# Autodesk Inventor assembly: 조립
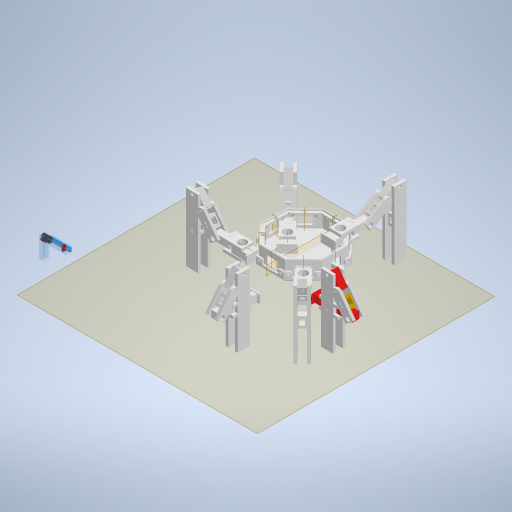
[picture p0: Inventor's stored thumbnail of the model, 512x512]
Saved by Autodesk Inventor 2024 (Build 280153000, 153)
## iProperties
Created: 2024-09-11
Part Number: 조립
Document SubType Name: Assembly
Designer: USER
Author: USER
## Documents named in this file (10)
- C:\Users\USER\Desktop\졸업작품\다리\조립.iam
- C:\Users\USER\Desktop\졸업작품\다리\다리 연결 부품-3.ipt
- C:\Users\USER\Desktop\졸업작품\다리\다리 프레임-0.ipt
- C:\Users\USER\Desktop\졸업작품\다리\다리 프레임-1.ipt
- C:\Users\USER\Desktop\졸업작품\다리\다리 프레임-2.ipt
- C:\Users\USER\Desktop\졸업작품\다리\다리 프레임-3.ipt
- C:\Users\USER\Desktop\졸업작품\다리\leg\LegTest.iam
- C:\Users\USER\Desktop\졸업작품\모터\모터.ipt
- C:\Users\USER\Desktop\졸업작품\다리\몸통.ipt
- C:\Users\USER\Desktop\졸업작품\다리\벽.ipt
## Components (76 placed, 9 different names)
1. 다리 연결 부품-3:1 — 메이트:12, 메이트:13, 메이트:14, 메이트:15, 메이트:25
2. 다리 프레임-0:1 — 메이트:3, 메이트:4, 메이트:11
3. 다리 프레임-1:1 — 메이트:3, 메이트:11, 메이트:16, 메이트:17, 메이트:39
4. 다리 프레임-2:1 — 메이트:12, 메이트:13, 메이트:22, 메이트:23, 메이트:25, 메이트:44, 메이트:46, 메이트:47
5. 다리 프레임-3:1 — 메이트:26, 메이트:27, 메이트:28, 메이트:48
6. 다리 프레임-1:2 — 메이트:4, 메이트:18, 메이트:19, 메이트:20
7. LegTest:1 [sub-assembly]
8. 모터:2 — 메이트:16, 메이트:17, 메이트:18, 메이트:19, 메이트:20, 메이트:21, 메이트:22, 메이트:23, 메이트:24, 메이트:39
9. 다리 프레임-2:2 — 메이트:14, 메이트:15, 메이트:21, 메이트:24
10. 다리 연결 부품-3:2 — 메이트:26, 메이트:27, 메이트:28, 메이트:29, 메이트:30, 메이트:31
11. 다리 프레임-3:2 — 메이트:29, 메이트:30, 메이트:31, 메이트:42, 메이트:45
12. 모터:3 — 메이트:42, 메이트:44, 메이트:45, 메이트:46, 메이트:47
13. 다리 연결 부품-3:3
14. 다리 프레임-0:2 — 메이트:208, 메이트:230, 메이트:231, 메이트:232
15. 다리 프레임-1:3 — 메이트:208
16. 다리 프레임-2:3
17. 다리 프레임-3:3 — 메이트:201
18. 다리 프레임-1:4
19. 모터:4
20. 다리 프레임-2:4
21. 다리 연결 부품-3:4
22. 다리 프레임-3:4
23. 모터:5
24. 다리 연결 부품-3:5
25. 다리 프레임-0:3
26. 다리 프레임-1:5
27. 다리 프레임-2:5
28. 다리 프레임-3:5 — 메이트:202, 메이트:206
29. 다리 프레임-1:6
30. 모터:6
31. 다리 프레임-2:6
32. 다리 연결 부품-3:6
33. 다리 프레임-3:6
34. 모터:7
35. 다리 연결 부품-3:7
36. 다리 프레임-0:4 — 메이트:211
37. 다리 프레임-1:7 — 메이트:211
38. 다리 프레임-2:7
39. 다리 프레임-3:7
40. 다리 프레임-1:8
41. 모터:8
42. 다리 프레임-2:8
43. 다리 연결 부품-3:8
44. 다리 프레임-3:8 — 메이트:204
45. 모터:9
46. 다리 연결 부품-3:9
47. 다리 프레임-0:5 — 메이트:212
48. 다리 프레임-1:9 — 메이트:212
49. 다리 프레임-2:9
50. 다리 프레임-3:9
51. 다리 프레임-1:10
52. 모터:10
53. 다리 프레임-2:10
54. 다리 연결 부품-3:10
55. 다리 프레임-3:10 — 메이트:203
56. 모터:11
57. 다리 연결 부품-3:11
58. 다리 프레임-0:6
59. 다리 프레임-1:11
60. 다리 프레임-2:11
61. 다리 프레임-3:11
62. 다리 프레임-1:12
63. 모터:12
64. 다리 프레임-2:12
65. 다리 연결 부품-3:12
66. 다리 프레임-3:12 — 메이트:205
67. 모터:13
68. 몸통:1 — 메이트:214, 메이트:215, 메이트:223, 메이트:224, 메이트:225, 메이트:226, 메이트:227, 메이트:228, 메이트:229, 플러쉬:8
69. 벽:1 — 메이트:214, 메이트:215, 메이트:216, 플러쉬:1
70. 벽:2 — 메이트:216, 플러쉬:1, 메이트:217, 플러쉬:2, 메이트:223
71. 벽:3 — 메이트:217, 플러쉬:2, 메이트:218, 플러쉬:3, 메이트:224
72. 벽:4 — 메이트:219, 플러쉬:4, 메이트:220, 플러쉬:5, 메이트:226
73. 벽:5 — 메이트:220, 플러쉬:5, 메이트:221, 플러쉬:6, 메이트:227, 플러쉬:8
74. 벽:6 — 메이트:218, 플러쉬:3, 메이트:219, 플러쉬:4, 메이트:225
75. 벽:7 — 메이트:221, 플러쉬:6, 메이트:222, 플러쉬:7, 메이트:228, 메이트:230, 메이트:231, 메이트:232
76. 벽:8 — 메이트:222, 플러쉬:7, 메이트:229
## Relationships (211: Mate 203, Flush 8)
- 메이트:3 [Mate]: 다리 프레임-0:1 ↔ 다리 프레임-1:1
- 메이트:4 [Mate]: 다리 프레임-0:1 ↔ 다리 프레임-1:2
- 메이트:11 [Mate]: 다리 프레임-0:1 ↔ 다리 프레임-1:1
- 메이트:12 [Mate]: 다리 연결 부품-3:1 ↔ 다리 프레임-2:1
- 메이트:13 [Mate]: 다리 연결 부품-3:1 ↔ 다리 프레임-2:1
- 메이트:14 [Mate]: 다리 연결 부품-3:1 ↔ 다리 프레임-2:2
- 메이트:15 [Mate]: 다리 연결 부품-3:1 ↔ 다리 프레임-2:2
- 메이트:16 [Mate]: 다리 프레임-1:1 ↔ 모터:2
- 메이트:17 [Mate]: 다리 프레임-1:1 ↔ 모터:2
- 메이트:18 [Mate]: 다리 프레임-1:2 ↔ 모터:2
- 메이트:19 [Mate]: 다리 프레임-1:2 ↔ 모터:2
- 메이트:20 [Mate]: 다리 프레임-1:2 ↔ 모터:2
- 메이트:21 [Mate]: 모터:2 ↔ 다리 프레임-2:2
- 메이트:22 [Mate]: 다리 프레임-2:1 ↔ 모터:2
- 메이트:23 [Mate]: 다리 프레임-2:1 ↔ 모터:2
- 메이트:24 [Mate]: 모터:2 ↔ 다리 프레임-2:2
- 메이트:25 [Mate]: 다리 연결 부품-3:1 ↔ 다리 프레임-2:1
- 메이트:26 [Mate]: 다리 프레임-3:1 ↔ 다리 연결 부품-3:2
- 메이트:27 [Mate]: 다리 프레임-3:1 ↔ 다리 연결 부품-3:2
- 메이트:28 [Mate]: 다리 프레임-3:1 ↔ 다리 연결 부품-3:2
- 메이트:29 [Mate]: 다리 연결 부품-3:2 ↔ 다리 프레임-3:2
- 메이트:30 [Mate]: 다리 연결 부품-3:2 ↔ 다리 프레임-3:2
- 메이트:31 [Mate]: 다리 연결 부품-3:2 ↔ 다리 프레임-3:2
- 메이트:39 [Mate]: 다리 프레임-1:1 ↔ 모터:2
- 메이트:42 [Mate]: 다리 프레임-3:2 ↔ 모터:3
- 메이트:44 [Mate]: 다리 프레임-2:1 ↔ 모터:3
- 메이트:45 [Mate]: 다리 프레임-3:2 ↔ 모터:3
- 메이트:46 [Mate]: 다리 프레임-2:1 ↔ 모터:3
- 메이트:47 [Mate]: 다리 프레임-2:1 ↔ 모터:3
- 메이트:48 [Mate]: 다리 프레임-3:1
- [Mate]: 다리 프레임-0:2 ↔ 다리 프레임-1:3
- [Mate]: 다리 프레임-0:2 ↔ 다리 프레임-1:4
- [Mate]: 다리 프레임-0:2 ↔ 다리 프레임-1:3
- [Mate]: 다리 연결 부품-3:3 ↔ 다리 프레임-2:3
- [Mate]: 다리 연결 부품-3:3 ↔ 다리 프레임-2:3
- [Mate]: 다리 연결 부품-3:3 ↔ 다리 프레임-2:4
- [Mate]: 다리 연결 부품-3:3 ↔ 다리 프레임-2:4
- [Mate]: 다리 프레임-1:3 ↔ 모터:4
- [Mate]: 다리 프레임-1:3 ↔ 모터:4
- [Mate]: 다리 프레임-1:4 ↔ 모터:4
- [Mate]: 다리 프레임-1:4 ↔ 모터:4
- [Mate]: 다리 프레임-1:4 ↔ 모터:4
- [Mate]: 모터:4 ↔ 다리 프레임-2:4
- [Mate]: 다리 프레임-2:3 ↔ 모터:4
- [Mate]: 다리 프레임-2:3 ↔ 모터:4
- [Mate]: 모터:4 ↔ 다리 프레임-2:4
- [Mate]: 다리 연결 부품-3:3 ↔ 다리 프레임-2:3
- [Mate]: 다리 프레임-3:3 ↔ 다리 연결 부품-3:4
- [Mate]: 다리 프레임-3:3 ↔ 다리 연결 부품-3:4
- [Mate]: 다리 프레임-3:3 ↔ 다리 연결 부품-3:4
- [Mate]: 다리 연결 부품-3:4 ↔ 다리 프레임-3:4
- [Mate]: 다리 연결 부품-3:4 ↔ 다리 프레임-3:4
- [Mate]: 다리 연결 부품-3:4 ↔ 다리 프레임-3:4
- [Mate]: 다리 프레임-1:3 ↔ 모터:4
- [Mate]: 다리 프레임-3:4 ↔ 모터:5
- [Mate]: 다리 프레임-2:3 ↔ 모터:5
- [Mate]: 다리 프레임-3:4 ↔ 모터:5
- [Mate]: 다리 프레임-2:3 ↔ 모터:5
- [Mate]: 다리 프레임-2:3 ↔ 모터:5
- [Mate]: 다리 프레임-0:3 ↔ 다리 프레임-1:5
- [Mate]: 다리 프레임-0:3 ↔ 다리 프레임-1:6
- [Mate]: 다리 프레임-0:3 ↔ 다리 프레임-1:5
- [Mate]: 다리 연결 부품-3:5 ↔ 다리 프레임-2:5
- [Mate]: 다리 연결 부품-3:5 ↔ 다리 프레임-2:5
- [Mate]: 다리 연결 부품-3:5 ↔ 다리 프레임-2:6
- [Mate]: 다리 연결 부품-3:5 ↔ 다리 프레임-2:6
- [Mate]: 다리 프레임-1:5 ↔ 모터:6
- [Mate]: 다리 프레임-1:5 ↔ 모터:6
- [Mate]: 다리 프레임-1:6 ↔ 모터:6
- [Mate]: 다리 프레임-1:6 ↔ 모터:6
- [Mate]: 다리 프레임-1:6 ↔ 모터:6
- [Mate]: 모터:6 ↔ 다리 프레임-2:6
- [Mate]: 다리 프레임-2:5 ↔ 모터:6
- [Mate]: 다리 프레임-2:5 ↔ 모터:6
- [Mate]: 모터:6 ↔ 다리 프레임-2:6
- [Mate]: 다리 연결 부품-3:5 ↔ 다리 프레임-2:5
- [Mate]: 다리 프레임-3:5 ↔ 다리 연결 부품-3:6
- [Mate]: 다리 프레임-3:5 ↔ 다리 연결 부품-3:6
- [Mate]: 다리 프레임-3:5 ↔ 다리 연결 부품-3:6
- [Mate]: 다리 연결 부품-3:6 ↔ 다리 프레임-3:6
- [Mate]: 다리 연결 부품-3:6 ↔ 다리 프레임-3:6
- [Mate]: 다리 연결 부품-3:6 ↔ 다리 프레임-3:6
- [Mate]: 다리 프레임-1:5 ↔ 모터:6
- [Mate]: 다리 프레임-3:6 ↔ 모터:7
- [Mate]: 다리 프레임-2:5 ↔ 모터:7
- [Mate]: 다리 프레임-3:6 ↔ 모터:7
- [Mate]: 다리 프레임-2:5 ↔ 모터:7
- [Mate]: 다리 프레임-2:5 ↔ 모터:7
- [Mate]: 다리 프레임-0:4 ↔ 다리 프레임-1:7
- [Mate]: 다리 프레임-0:4 ↔ 다리 프레임-1:8
- [Mate]: 다리 프레임-0:4 ↔ 다리 프레임-1:7
- [Mate]: 다리 연결 부품-3:7 ↔ 다리 프레임-2:7
- [Mate]: 다리 연결 부품-3:7 ↔ 다리 프레임-2:7
- [Mate]: 다리 연결 부품-3:7 ↔ 다리 프레임-2:8
- [Mate]: 다리 연결 부품-3:7 ↔ 다리 프레임-2:8
- [Mate]: 다리 프레임-1:7 ↔ 모터:8
- [Mate]: 다리 프레임-1:7 ↔ 모터:8
- [Mate]: 다리 프레임-1:8 ↔ 모터:8
- [Mate]: 다리 프레임-1:8 ↔ 모터:8
- [Mate]: 다리 프레임-1:8 ↔ 모터:8
- [Mate]: 모터:8 ↔ 다리 프레임-2:8
- [Mate]: 다리 프레임-2:7 ↔ 모터:8
- [Mate]: 다리 프레임-2:7 ↔ 모터:8
- [Mate]: 모터:8 ↔ 다리 프레임-2:8
- [Mate]: 다리 연결 부품-3:7 ↔ 다리 프레임-2:7
- [Mate]: 다리 프레임-3:7 ↔ 다리 연결 부품-3:8
- [Mate]: 다리 프레임-3:7 ↔ 다리 연결 부품-3:8
- [Mate]: 다리 프레임-3:7 ↔ 다리 연결 부품-3:8
- [Mate]: 다리 연결 부품-3:8 ↔ 다리 프레임-3:8
- [Mate]: 다리 연결 부품-3:8 ↔ 다리 프레임-3:8
- [Mate]: 다리 연결 부품-3:8 ↔ 다리 프레임-3:8
- [Mate]: 다리 프레임-1:7 ↔ 모터:8
- [Mate]: 다리 프레임-3:8 ↔ 모터:9
- [Mate]: 다리 프레임-2:7 ↔ 모터:9
- [Mate]: 다리 프레임-3:8 ↔ 모터:9
- [Mate]: 다리 프레임-2:7 ↔ 모터:9
- [Mate]: 다리 프레임-2:7 ↔ 모터:9
- [Mate]: 다리 프레임-0:5 ↔ 다리 프레임-1:9
- [Mate]: 다리 프레임-0:5 ↔ 다리 프레임-1:10
- [Mate]: 다리 프레임-0:5 ↔ 다리 프레임-1:9
- [Mate]: 다리 연결 부품-3:9 ↔ 다리 프레임-2:9
- [Mate]: 다리 연결 부품-3:9 ↔ 다리 프레임-2:9
- [Mate]: 다리 연결 부품-3:9 ↔ 다리 프레임-2:10
- [Mate]: 다리 연결 부품-3:9 ↔ 다리 프레임-2:10
- [Mate]: 다리 프레임-1:9 ↔ 모터:10
- [Mate]: 다리 프레임-1:9 ↔ 모터:10
- [Mate]: 다리 프레임-1:10 ↔ 모터:10
- [Mate]: 다리 프레임-1:10 ↔ 모터:10
- [Mate]: 다리 프레임-1:10 ↔ 모터:10
- [Mate]: 모터:10 ↔ 다리 프레임-2:10
- [Mate]: 다리 프레임-2:9 ↔ 모터:10
- [Mate]: 다리 프레임-2:9 ↔ 모터:10
- [Mate]: 모터:10 ↔ 다리 프레임-2:10
- [Mate]: 다리 연결 부품-3:9 ↔ 다리 프레임-2:9
- [Mate]: 다리 프레임-3:9 ↔ 다리 연결 부품-3:10
- [Mate]: 다리 프레임-3:9 ↔ 다리 연결 부품-3:10
- [Mate]: 다리 프레임-3:9 ↔ 다리 연결 부품-3:10
- [Mate]: 다리 연결 부품-3:10 ↔ 다리 프레임-3:10
- [Mate]: 다리 연결 부품-3:10 ↔ 다리 프레임-3:10
- [Mate]: 다리 연결 부품-3:10 ↔ 다리 프레임-3:10
- [Mate]: 다리 프레임-1:9 ↔ 모터:10
- [Mate]: 다리 프레임-3:10 ↔ 모터:11
- [Mate]: 다리 프레임-2:9 ↔ 모터:11
- [Mate]: 다리 프레임-3:10 ↔ 모터:11
- [Mate]: 다리 프레임-2:9 ↔ 모터:11
- [Mate]: 다리 프레임-2:9 ↔ 모터:11
- [Mate]: 다리 프레임-0:6 ↔ 다리 프레임-1:11
- [Mate]: 다리 프레임-0:6 ↔ 다리 프레임-1:12
- [Mate]: 다리 프레임-0:6 ↔ 다리 프레임-1:11
- [Mate]: 다리 연결 부품-3:11 ↔ 다리 프레임-2:11
- [Mate]: 다리 연결 부품-3:11 ↔ 다리 프레임-2:11
- [Mate]: 다리 연결 부품-3:11 ↔ 다리 프레임-2:12
- [Mate]: 다리 연결 부품-3:11 ↔ 다리 프레임-2:12
- [Mate]: 다리 프레임-1:11 ↔ 모터:12
- [Mate]: 다리 프레임-1:11 ↔ 모터:12
- [Mate]: 다리 프레임-1:12 ↔ 모터:12
- [Mate]: 다리 프레임-1:12 ↔ 모터:12
- [Mate]: 다리 프레임-1:12 ↔ 모터:12
- [Mate]: 모터:12 ↔ 다리 프레임-2:12
- [Mate]: 다리 프레임-2:11 ↔ 모터:12
- [Mate]: 다리 프레임-2:11 ↔ 모터:12
- [Mate]: 모터:12 ↔ 다리 프레임-2:12
- [Mate]: 다리 연결 부품-3:11 ↔ 다리 프레임-2:11
- [Mate]: 다리 프레임-3:11 ↔ 다리 연결 부품-3:12
- [Mate]: 다리 프레임-3:11 ↔ 다리 연결 부품-3:12
- [Mate]: 다리 프레임-3:11 ↔ 다리 연결 부품-3:12
- [Mate]: 다리 연결 부품-3:12 ↔ 다리 프레임-3:12
- [Mate]: 다리 연결 부품-3:12 ↔ 다리 프레임-3:12
- [Mate]: 다리 연결 부품-3:12 ↔ 다리 프레임-3:12
- [Mate]: 다리 프레임-1:11 ↔ 모터:12
- [Mate]: 다리 프레임-3:12 ↔ 모터:13
- [Mate]: 다리 프레임-2:11 ↔ 모터:13
- [Mate]: 다리 프레임-3:12 ↔ 모터:13
- [Mate]: 다리 프레임-2:11 ↔ 모터:13
- [Mate]: 다리 프레임-2:11 ↔ 모터:13
- 메이트:201 [Mate]: 다리 프레임-3:3
- 메이트:202 [Mate]: 다리 프레임-3:5
- 메이트:203 [Mate]: 다리 프레임-3:10
- 메이트:204 [Mate]: 다리 프레임-3:8
- 메이트:205 [Mate]: 다리 프레임-3:12
- 메이트:206 [Mate]: 다리 프레임-3:5
- 메이트:208 [Mate]: 다리 프레임-0:2 ↔ 다리 프레임-1:3
- 메이트:211 [Mate]: 다리 프레임-0:4 ↔ 다리 프레임-1:7
- 메이트:212 [Mate]: 다리 프레임-0:5 ↔ 다리 프레임-1:9
- 메이트:214 [Mate]: 몸통:1 ↔ 벽:1
- 메이트:215 [Mate]: 몸통:1 ↔ 벽:1
- 메이트:216 [Mate]: 벽:1 ↔ 벽:2
- 플러쉬:1 [Flush]: 벽:1 ↔ 벽:2
- 메이트:217 [Mate]: 벽:2 ↔ 벽:3
- 플러쉬:2 [Flush]: 벽:2 ↔ 벽:3
- 메이트:218 [Mate]: 벽:3 ↔ 벽:6
- 플러쉬:3 [Flush]: 벽:3 ↔ 벽:6
- 메이트:219 [Mate]: 벽:4 ↔ 벽:6
- 플러쉬:4 [Flush]: 벽:4 ↔ 벽:6
- 메이트:220 [Mate]: 벽:4 ↔ 벽:5
- 플러쉬:5 [Flush]: 벽:4 ↔ 벽:5
- 메이트:221 [Mate]: 벽:5 ↔ 벽:7
- 플러쉬:6 [Flush]: 벽:5 ↔ 벽:7
- 메이트:222 [Mate]: 벽:7 ↔ 벽:8
- 플러쉬:7 [Flush]: 벽:7 ↔ 벽:8
- 메이트:223 [Mate]: 몸통:1 ↔ 벽:2
- 메이트:224 [Mate]: 몸통:1 ↔ 벽:3
- 메이트:225 [Mate]: 몸통:1 ↔ 벽:6
- 메이트:226 [Mate]: 몸통:1 ↔ 벽:4
- 메이트:227 [Mate]: 몸통:1 ↔ 벽:5
- 메이트:228 [Mate]: 몸통:1 ↔ 벽:7
- 메이트:229 [Mate]: 몸통:1 ↔ 벽:8
- 플러쉬:8 [Flush]: 몸통:1 ↔ 벽:5
- 메이트:230 [Mate]: 다리 프레임-0:2 ↔ 벽:7
- 메이트:231 [Mate]: 다리 프레임-0:2 ↔ 벽:7
- 메이트:232 [Mate]: 다리 프레임-0:2 ↔ 벽:7
## Named parameters: d49_d3 = 0 mm, d50_d4 = 0 mm, d51_d11 = 0 mm, d52_d12 = 0 mm, d53_d13 = 0 mm, d54_d14 = 0 mm, d55_d15 = 0 mm, d56_d16 = 0 mm, d57_d17 = 0 mm, d58_d18 = 0 mm, d59_d19 = 0 mm, d60_d20 = 0 mm, d61_d21 = 0 mm, d62_d22 = 0 mm, d63_d23 = 0 mm, d64_d24 = 0 mm, d65_d25 = 0 mm, d66_d26 = 0 mm, d67_d27 = 0 mm, d68_d28 = 0 mm, d69_d29 = 0 mm, d70_d30 = 0 mm, d71_d31 = 0 mm, d72_d39 = 0 mm, d73_d42 = 0 mm, d74_d44 = 0 mm, d75_d45 = 0 mm, d76_d46 = 0 mm, d77_d47 = 0 mm, d78_d3 = 0 mm, d79_d4 = 0 mm, d80_d11 = 0 mm, d81_d12 = 0 mm, d82_d13 = 0 mm, d83_d14 = 0 mm, d84_d15 = 0 mm, d85_d16 = 0 mm, d86_d17 = 0 mm, d87_d18 = 0 mm, d88_d19 = 0 mm, d89_d20 = 0 mm, d90_d21 = 0 mm, d91_d22 = 0 mm, d92_d23 = 0 mm, d93_d24 = 0 mm, d94_d25 = 0 mm, d95_d26 = 0 mm, d96_d27 = 0 mm, d97_d28 = 0 mm, d98_d29 = 0 mm, d99_d30 = 0 mm, d100_d31 = 0 mm, d101_d39 = 0 mm, d102_d42 = 0 mm, d103_d44 = 0 mm, d104_d45 = 0 mm, d105_d46 = 0 mm, d106_d47 = 0 mm, d107_d3 = 0 mm, d108_d4 = 0 mm, d109_d11 = 0 mm, d110_d12 = 0 mm, d111_d13 = 0 mm, d112_d14 = 0 mm, d113_d15 = 0 mm, d114_d16 = 0 mm, d115_d17 = 0 mm, d116_d18 = 0 mm, d117_d19 = 0 mm, d118_d20 = 0 mm, d119_d21 = 0 mm, d120_d22 = 0 mm, d121_d23 = 0 mm, d122_d24 = 0 mm, d123_d25 = 0 mm, d124_d26 = 0 mm, d125_d27 = 0 mm, d126_d28 = 0 mm, d127_d29 = 0 mm, d128_d30 = 0 mm, d129_d31 = 0 mm, d130_d39 = 0 mm, d131_d42 = 0 mm, d132_d44 = 0 mm, d133_d45 = 0 mm, d134_d46 = 0 mm, d135_d47 = 0 mm, d136_d3 = 0 mm, d137_d4 = 0 mm, d138_d11 = 0 mm, d139_d12 = 0 mm, d140_d13 = 0 mm, d141_d14 = 0 mm, d142_d15 = 0 mm, d143_d16 = 0 mm, d144_d17 = 0 mm, d145_d18 = 0 mm, d146_d19 = 0 mm, d147_d20 = 0 mm, d148_d21 = 0 mm, d149_d22 = 0 mm, d150_d23 = 0 mm, d151_d24 = 0 mm, d152_d25 = 0 mm, d153_d26 = 0 mm, d154_d27 = 0 mm, d155_d28 = 0 mm, d156_d29 = 0 mm, d157_d30 = 0 mm, d158_d31 = 0 mm, d159_d39 = 0 mm, d160_d42 = 0 mm, d161_d44 = 0 mm, d162_d45 = 0 mm, d163_d46 = 0 mm, d164_d47 = 0 mm, d165_d3 = 0 mm, d166_d4 = 0 mm, d167_d11 = 0 mm, d168_d12 = 0 mm, d169_d13 = 0 mm, d170_d14 = 0 mm, d171_d15 = 0 mm, d172_d16 = 0 mm, d173_d17 = 0 mm, d174_d18 = 0 mm, d175_d19 = 0 mm, d176_d20 = 0 mm, d177_d21 = 0 mm, d178_d22 = 0 mm, d179_d23 = 0 mm, d180_d24 = 0 mm, d181_d25 = 0 mm, d182_d26 = 0 mm, d183_d27 = 0 mm, d184_d28 = 0 mm, d185_d29 = 0 mm, d186_d30 = 0 mm, d187_d31 = 0 mm, d188_d39 = 0 mm, d189_d42 = 0 mm, d190_d44 = 0 mm, d191_d45 = 0 mm, d192_d46 = 0 mm, d193_d47 = 0 mm
